# Autodesk Inventor assembly: skrzydlo_ster
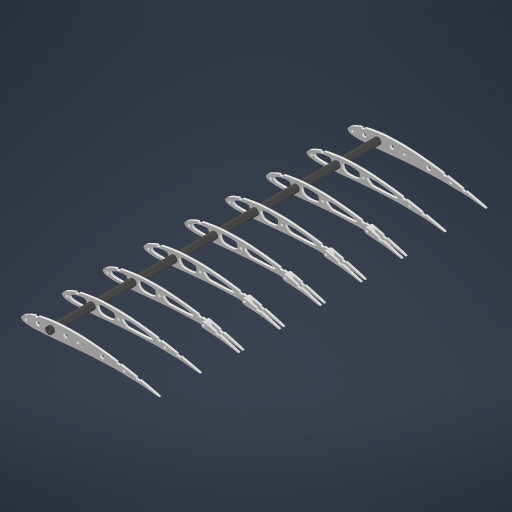
[picture p0: Inventor's stored thumbnail of the model, 512x512]
Saved by Autodesk Inventor 2023 (Build 270158000, 158)
## iProperties
Created: 2023-01-05
Part Number: skrzydlo_ster
Document SubType Name: Assembly
Designer: szykr
Author: szykr
## Documents named in this file (5)
- D:\Folder Instalacyjny\GitHub Pliki\Solaris\new model\skrzydlo_ster.iam
- D:\Folder Instalacyjny\GitHub Pliki\Solaris\new model\Wingspar trochemniejnizpol metrowy.ipt
- D:\Folder Instalacyjny\GitHub Pliki\Solaris\new model\Żerbo montaż.ipt
- D:\Folder Instalacyjny\GitHub Pliki\Solaris\new model\Zebro_lotka.iam
- D:\Folder Instalacyjny\GitHub Pliki\Solaris\new model\Żebro default.ipt
## Components (10 placed, 4 different names)
1. Wingspar trochemniejnizpol metrowy:1 — Insert:1
2. Żerbo montaż:1 — Insert:1, Insert:3, Insert:4, Insert:5, Insert:6
3. Żerbo montaż:2 — Insert:6
4. Żebro default:3 — Insert:5
5. Zebro_lotka:1 [sub-assembly] — Insert:3
6. Zebro_lotka:2 [sub-assembly]
7. Zebro_lotka:3 [sub-assembly]
8. Zebro_lotka:4 [sub-assembly]
9. Zebro_lotka:5 [sub-assembly]
10. Żebro default:1 — Insert:4
## Component patterns: Component Pattern 1:1 (1 elements), (5 elements, first: Zebro_lotka:1), (1 elements, first: Żebro default:1)
## Relationships (5: Insert 5)
- Insert:1 (8.57 mm): Wingspar trochemniejnizpol metrowy:1 ↔ Żerbo montaż:1
- Insert:3 (118.1075 mm): Żerbo montaż:1 ↔ Zebro_lotka:1
- Insert:4 (413.3763 mm): Żerbo montaż:1 ↔ Żebro default:1
- Insert:5 (59.0538 mm): Żerbo montaż:1 ↔ Żebro default:3
- Insert:6 (472.43 mm): Żerbo montaż:1 ↔ Żerbo montaż:2
## Named parameters: dlugosc = 472.43 mm, pre_zebra = 1, post_zebra = 1, lotki = 5, ilosc_zeber = 8, spacing = 59.05375 mm
